# Autodesk Inventor assembly: bio-roter inductive charger
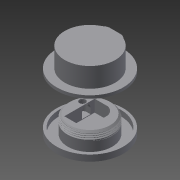
[picture p0: Inventor's stored thumbnail of the model, 180x180]
Saved by Autodesk Inventor 2017 (Build 210142000, 142)
## iProperties
Created: 2016-09-02
Part Number: bio-roter inductive charger
Document SubType Name: Assembly
Designer: Dmitry
Author: Dmitry
## Documents named in this file (3)
- C:\Users\Dmitry\Documents\GitHub\HARDWARE\bio-roter_charger\bio-roter inductive charger.iam
- C:\Users\Dmitry\Documents\GitHub\HARDWARE\bio-roter_charger\TX_face].ipt
- C:\Users\Dmitry\Documents\GitHub\HARDWARE\bio-roter_charger\TX_case.ipt
## Components (2 placed, 2 different names)
1. TX_face]:1 — Mate:1
2. TX_case:1 — Mate:1, Mate:2
## Relationships (2: Mate 2)
- Mate:1: TX_face]:1 ↔ TX_case:1
- Mate:2: TX_case:1
